# Autodesk Inventor assembly: PS20025
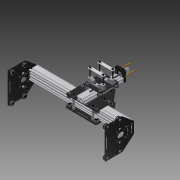
[picture p0: Inventor's stored thumbnail of the model, 180x180]
Saved by Autodesk Inventor 2014 (Build 180170000, 170)
## iProperties
Created: 2013-09-18
Part Number: PS20025
Document SubType Name: Assembly
Designer: Edward
Author: Edward
## Documents named in this file (3)
- C:\Users\Edward\Documents\GitHub\Shapeoko_2\Autodesk_Inventor_Project\PS20025.iam
- C:\Users\Edward\Documents\GitHub\Shapeoko_2\Autodesk_Inventor_Project\PS20023.iam
- C:\Users\Edward\Documents\GitHub\Shapeoko_2\Autodesk_Inventor_Project\PS20027.iam
## Components (2 placed, 2 different names)
1. PS20023:1 [sub-assembly] — Mate:1, Flush:1
2. PS20027:1 [sub-assembly] — Mate:1, Flush:1
## Relationships (2: Mate 1, Flush 1)
- Mate:1 (6.35 mm): PS20023:1 ↔ PS20027:1
- Flush:1 (-25 mm): PS20023:1 ↔ PS20027:1
